# Autodesk Inventor assembly: pcbIOExt
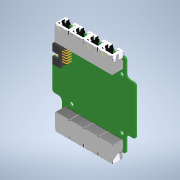
[picture p0: Inventor's stored thumbnail of the model, 180x180]
Saved by Autodesk Inventor 2021 (Build 250183000, 183)
## iProperties
Created: 2023-08-07
Part Number: pcbIOExt
Document SubType Name: Assembly
Designer: michal
Author: michal
## Documents named in this file (4)
- C:\Users\micha\OneDrive\Dokumenty\GitHub\escape_room_hw_v2\Enclosure\pcbIOExt.iam
- C:\Users\micha\OneDrive\Dokumenty\GitHub\escape_room_hw_v2\Enclosure\pcbIO.ipt
- C:\Users\micha\OneDrive\Dokumenty\GitHub\escape_room_hw_v2\Enclosure\Commercial\rjPack.iam
- C:\Users\micha\Downloads\612010235221.iam
## Components (4 placed, 3 different names)
1. pcbIO:1 — Mate:1, Flush:1, Mate:2, Flush:2, Mate:3, Mate:4, Flush:4, Flush:5
2. rjPack:1 [sub-assembly] — Mate:1, Flush:1, Flush:3
3. rjPack:2 [sub-assembly] — Mate:2, Flush:2, Flush:3, Flush:5
4. 612010235221:1 [sub-assembly] — Mate:3, Mate:4, Flush:4
## Relationships (9: Flush 5, Mate 4)
- Mate:1: pcbIO:1 ↔ rjPack:1
- Flush:1 (-6 mm): pcbIO:1 ↔ rjPack:1
- Mate:2: pcbIO:1 ↔ rjPack:2
- Flush:2 (-6 mm): pcbIO:1 ↔ rjPack:2
- Flush:3: rjPack:1 ↔ rjPack:2
- Mate:3: pcbIO:1 ↔ 612010235221:1
- Mate:4 (-1 mm): pcbIO:1 ↔ 612010235221:1
- Flush:4 (-2 mm): pcbIO:1 ↔ 612010235221:1
- Flush:5 (3.6 mm): pcbIO:1 ↔ rjPack:2
